# Autodesk Inventor assembly: UltrasonicSensor2
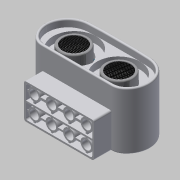
[picture p0: Inventor's stored thumbnail of the model, 180x180]
Saved by Autodesk Inventor 2019.3 (Build 233278000, 278)
## iProperties
Created: 2019-02-04
Part Number: UltrasonicSensor2
Document SubType Name: Assembly
Designer: Varga Daniel
Sending System: SolidWorks 2018
Last Author: david
Last Saved: 2019-02-07
Author: Varga Daniel
## Documents named in this file (4)
- C:\!_Dani\!_cloud\OneDrive\!_munka\Revolution\RevvyDemoKit\Structural parts\Demo parts\Ultrasonic sensor\Inventor imported\UltrasonicSensor2_ver2.iam
- C:\!_Dani\!_cloud\OneDrive\!_munka\Revolution\RevvyDemoKit\Structural parts\Demo parts\Ultrasonic sensor\Inventor imported\HC-SR04.ipt
- C:\!_Dani\!_cloud\OneDrive\!_munka\Revolution\RevvyDemoKit\Structural parts\Demo parts\Ultrasonic sensor\Inventor imported\rj45_vert.ipt
- C:\!_Dani\!_cloud\OneDrive\!_munka\Revolution\RevvyDemoKit\Structural parts\Demo parts\Ultrasonic sensor\Inventor imported\UScA_ver2.ipt
## Components (3 placed, 3 different names)
1. HC-SR04:1 — Mate:2, Angle:2, Flush:3, Mate:3
2. rj45_vert:1 — Flush:1, Mate:3, Mate:4, Angle:3
3. UScA_ver2:1 — Flush:1, Mate:1, Angle:1, Flush:3
## Relationships (11: Mate 5, Flush 3, Angle 3)
- Flush:1 (-2 mm): rj45_vert:1 ↔ UScA_ver2:1
- Mate:1: UScA_ver2:1
- Angle:1 (0 deg): UScA_ver2:1
- Mate:2: HC-SR04:1
- Angle:2 (0 deg): HC-SR04:1
- Flush:2
- Flush:3 (5.939 mm): HC-SR04:1 ↔ UScA_ver2:1
- Mate:3: HC-SR04:1 ↔ rj45_vert:1
- Mate:4 (0.5 mm): rj45_vert:1
- Angle:3 (0 deg): rj45_vert:1
- Mate:5
